# Autodesk Inventor assembly: FE-00018
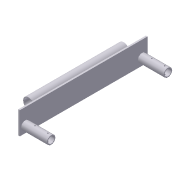
[picture p0: Inventor's stored thumbnail of the model, 180x180]
Saved by Autodesk Inventor 2012 (Build 160160000, 160)
## iProperties
Company: FIRST
Created: 2008-05-30
Part Number: FE-00018
Document SubType Name: Weldment
Designer: dfoster
Weld Material: Welded Aluminum-6061
Description: Corner Connector
Title: Corner Connector
Author: dfoster
## Documents named in this file (5)
- C:\Data Folder\FRC 2012 Field\Components\FE-00018.iam
- C:\Data Folder\FRC 2012 Field\Components\FE-00018-01.ipt
- C:\Data Folder\FRC 2012 Field\Components\FE-00018-02.ipt
- C:\Data Folder\FRC 2012 Field\Components\FE-00018-03.ipt
- C:\Data Folder\FRC 2012 Field\Components\FE-00018-04.ipt
## Components (5 placed, 4 different names)
1. FE-00018-01:1 — Tangent:1, Flush:1, Tangent:2, Flush:2
2. FE-00018-02:1 — Mate:2, Tangent:5, Tangent:6
3. FE-00018-02:2 — Mate:1, Tangent:3, Tangent:4
4. FE-00018-03:1 — Tangent:1, Flush:1, Angle:1, Tangent:2, Mate:1, Mate:2, Tangent:3, Tangent:4, Tangent:5, Tangent:6, Mate:3, Flush:3
5. FE-00018-04:1 — Mate:3, Flush:2, Flush:3
## Relationships (13: Tangent 6, Flush 3, Mate 3, Angle 1)
- Tangent:1 (2.3813 mm): FE-00018-01:1 ↔ FE-00018-03:1
- Flush:1 (-63.5 mm): FE-00018-01:1 ↔ FE-00018-03:1
- Angle:1 (0 deg): FE-00018-03:1
- Tangent:2 (2.3813 mm): FE-00018-01:1 ↔ FE-00018-03:1
- Mate:1: FE-00018-02:2 ↔ FE-00018-03:1
- Mate:2: FE-00018-02:1 ↔ FE-00018-03:1
- Tangent:3 (4.7625 mm): FE-00018-02:2 ↔ FE-00018-03:1
- Tangent:4 (11.1125 mm): FE-00018-02:2 ↔ FE-00018-03:1
- Tangent:5 (11.1125 mm): FE-00018-02:1 ↔ FE-00018-03:1
- Tangent:6 (4.7625 mm): FE-00018-02:1 ↔ FE-00018-03:1
- Mate:3: FE-00018-03:1 ↔ FE-00018-04:1
- Flush:2: FE-00018-01:1 ↔ FE-00018-04:1
- Flush:3 (17.0688 mm): FE-00018-03:1 ↔ FE-00018-04:1
